# Autodesk Inventor assembly: Joint Assembly
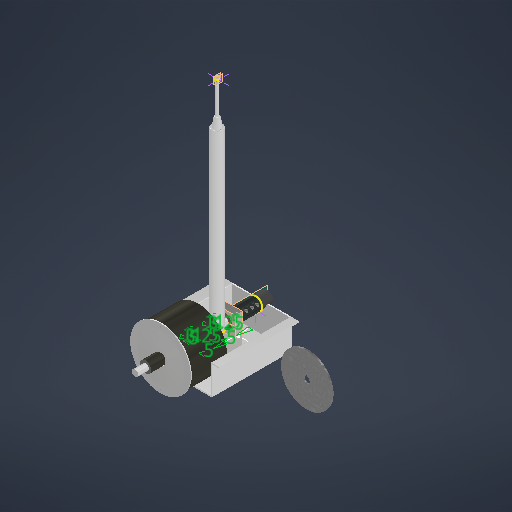
[picture p0: Inventor's stored thumbnail of the model, 512x512]
Saved by Autodesk Inventor 2026.3 (Build 303398000, 398)
## iProperties
Created: 2026-07-22
Part Number: Joint Assembly
Document SubType Name: Assembly
Designer: matot
Author: matot
## Documents named in this file (14)
- C:\Users\matot\OneDrive - Stellenbosch University\2026\MechatronicsProject478\Building the joint\Joint Assembly\Joint Assembly.iam
- C:\Users\matot\OneDrive - Stellenbosch University\2026\MechatronicsProject478\Building the joint\Joint Assembly\Brake disc.ipt
- C:\Users\matot\OneDrive - Stellenbosch University\2026\MechatronicsProject478\Building the joint\Joint Assembly\Electromagnet.iam
- C:\Users\matot\OneDrive - Stellenbosch University\2026\MechatronicsProject478\Building the joint\Joint Assembly\2058786.iam
- C:\Users\matot\OneDrive - Stellenbosch University\2026\MechatronicsProject478\Building the joint\Joint Assembly\mclx-20-20-f.iam
- C:\Users\matot\OneDrive - Stellenbosch University\2026\MechatronicsProject478\Building the joint\Joint Assembly\Reducer bushing.ipt
- C:\Users\matot\OneDrive - Stellenbosch University\2026\MechatronicsProject478\Building the joint\Joint Assembly\Optical Encoder.ipt
- C:\Users\matot\OneDrive - Stellenbosch University\2026\MechatronicsProject478\Building the joint\Joint Assembly\Rough draft shaft.ipt
- C:\Users\matot\OneDrive - Stellenbosch University\2026\MechatronicsProject478\Building the joint\Joint Assembly\8236976.ipt
- C:\Users\matot\OneDrive - Stellenbosch University\2026\MechatronicsProject478\Building the joint\Joint Assembly\Output Link.iam
- C:\Users\matot\OneDrive - Stellenbosch University\2026\MechatronicsProject478\Building the joint\Joint Assembly\Bearing housing bottom.ipt
- C:\Users\matot\OneDrive - Stellenbosch University\2026\MechatronicsProject478\Building the joint\Joint Assembly\Bearing housing top.ipt
- C:\Users\matot\OneDrive - Stellenbosch University\2026\MechatronicsProject478\Building the joint\Joint Assembly\Joint Housing Bottom.iam
- C:\Users\matot\OneDrive - Stellenbosch University\2026\MechatronicsProject478\Building the joint\Joint Assembly\Prressure plate.ipt
## Components (17 placed, 13 different names)
1. Brake disc:1
2. Electromagnet:1 [sub-assembly] — Insert:18, Tangent:1, Tangent:2, Flush:1, Insert:23
3. 2058786:1 [sub-assembly] — Insert:11, Insert:12, Insert:21
4. 2058786:2 [sub-assembly] — Insert:10, Insert:13, Insert:15, Insert:20
5. mclx-20-20-f:1 [sub-assembly] — Mate:1, Insert:19
6. Reducer bushing:2 — Insert:2, Mate:1
7. Optical Encoder:1 — Insert:2, Insert:17, Insert:19
8. 8236976:1 — Insert:12, Insert:18
9. 8236976:2 — Insert:13
10. Output Link:1 [sub-assembly] — Mate:2, Mate:3, Insert:10, Insert:11
11. Rough draft shaft:1 — Mate:2, Mate:3, Insert:17
12. Bearing housing bottom:1 — Insert:21, Insert:22
13. Bearing housing bottom:2 — Insert:15
14. Bearing housing top:2 — Insert:22
15. Bearing housing top:3 — Insert:20
16. Joint Housing Bottom:1 [sub-assembly] — Tangent:1, Tangent:2, Flush:1
17. Prressure plate:1 — Insert:23
## Relationships (19: Insert 13, Mate 3, Tangent 2, Flush 1)
- Insert:2: Reducer bushing:2 ↔ Optical Encoder:1
- Mate:1: mclx-20-20-f:1 ↔ Reducer bushing:2
- Mate:2: Output Link:1 ↔ Rough draft shaft:1
- Mate:3: Output Link:1 ↔ Rough draft shaft:1
- Insert:10: 2058786:2 ↔ Output Link:1
- Insert:11: 2058786:1 ↔ Output Link:1
- Insert:12: 2058786:1 ↔ 8236976:1
- Insert:13: 2058786:2 ↔ 8236976:2
- Insert:15: 2058786:2 ↔ Bearing housing bottom:2
- Insert:17: Optical Encoder:1 ↔ Rough draft shaft:1
- Insert:18: Electromagnet:1 ↔ 8236976:1
- Insert:19: mclx-20-20-f:1 ↔ Optical Encoder:1
- Tangent:1: Electromagnet:1 ↔ Joint Housing Bottom:1
- Tangent:2: Electromagnet:1 ↔ Joint Housing Bottom:1
- Flush:1 (-65 mm): Electromagnet:1 ↔ Joint Housing Bottom:1
- Insert:20: 2058786:2 ↔ Bearing housing top:3
- Insert:21: 2058786:1 ↔ Bearing housing bottom:1
- Insert:22: Bearing housing bottom:1 ↔ Bearing housing top:2
- Insert:23: Electromagnet:1 ↔ Prressure plate:1
